# Autodesk Inventor assembly: z idler pulley
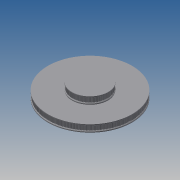
[picture p0: Inventor's stored thumbnail of the model, 180x180]
Saved by Autodesk Inventor 2013 (Build 170138000, 138)
## iProperties
Created: 2017-03-30
Part Number: z idler pulley
Document SubType Name: Assembly
Designer: employee
Author: employee
## Documents named in this file (3)
- C:\Users\employee\Desktop\SCARA\z idler pulley.iam
- C:\Users\employee\Desktop\SCARA\235 pulley blank.ipt
- C:\Users\employee\Desktop\SCARA\100 pulley blank.ipt
## Components (2 placed, 2 different names)
1. 235 pulley blank:1 — Insert:1, Mate:1
2. 100 pulley blank:1 — Insert:1, Mate:1
## Relationships (2: Insert 1, Mate 1)
- Insert:1: 235 pulley blank:1 ↔ 100 pulley blank:1
- Mate:1: 235 pulley blank:1 ↔ 100 pulley blank:1
